# Autodesk Inventor assembly: NewClawArm
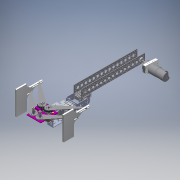
[picture p0: Inventor's stored thumbnail of the model, 180x180]
Saved by Autodesk Inventor 2017 (Build 210142000, 142)
## iProperties
Created: 2018-01-16
Part Number: NewClawArm
Document SubType Name: Assembly
Designer: User
Author: User
## Documents named in this file (6)
- C:\Robotics\CAD\2017-18_CAD\Miscellaneous\NewClawArm.iam
- C:\Robotics\CAD\COTSParts\Actobotics\585 parts\585454.ipt
- C:\Robotics\CAD\2017-18_CAD\Claw2017-18.iam
- C:\Robotics\CAD\COTSParts\Motors\Andymark 2964  NeveRest 40 Motor.ipt
- C:\Robotics\CAD\COTSParts\Tetrix\tetrix-motor-mounts-1.snapshot.1\Tetrex 2pc motor mount.ipt
- C:\Robotics\CAD\COTSParts\Tetrix\Tetrix hub - motor.ipt
## Components (5 placed, 5 different names)
1. 585454:1 — Mate:1, Mate:2, Mate:6, Mate:7
2. Claw2017-18:1 [sub-assembly] — Mate:1, Mate:2
3. Andymark 2964  NeveRest 40 Motor:1 — Mate:3, Mate:4, Mate:5, Flush:1
4. Tetrex 2pc motor mount:1 — Mate:3, Mate:4
5. Tetrix hub - motor:1 — Mate:5, Flush:1, Mate:6, Mate:7
## Relationships (8: Mate 7, Flush 1)
- Mate:1: 585454:1 ↔ Claw2017-18:1
- Mate:2: 585454:1 ↔ Claw2017-18:1
- Mate:3: Andymark 2964  NeveRest 40 Motor:1 ↔ Tetrex 2pc motor mount:1
- Mate:4: Andymark 2964  NeveRest 40 Motor:1 ↔ Tetrex 2pc motor mount:1
- Mate:5: Andymark 2964  NeveRest 40 Motor:1 ↔ Tetrix hub - motor:1
- Flush:1: Andymark 2964  NeveRest 40 Motor:1 ↔ Tetrix hub - motor:1
- Mate:6: 585454:1 ↔ Tetrix hub - motor:1
- Mate:7: 585454:1 ↔ Tetrix hub - motor:1
